# Autodesk Inventor assembly: Right_Upper_Engine_Mount_Rod_Assembly_V1
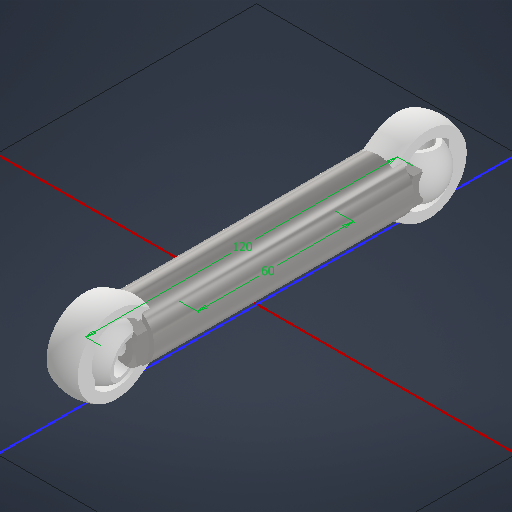
[picture p0: Inventor's stored thumbnail of the model, 512x512]
Saved by Autodesk Inventor 2026.1 (Build 301233000, 233)
## iProperties
Created: 2026-07-28
Part Number: Right_Upper_Engine_Mount_Rod_Assembly_V1
Document SubType Name: Assembly
Designer: share
_SolveAssemblyDoc: Frame Generator Solve Assembly
_Version: 15.0.0
Author: share
## iProperties of the stored document MemberDocs/xWu1g1ya3Psmt1s4v2xjpsksqJb
_SolveAssemblyDoc: Frame Generator Solve Assembly
_Version: 15.0.0
Created: 2026-07-28
Part Number: Right_Upper_Engine_Mount_Rod_Assembly_V1
Document SubType Name: Assembly
Designer: share
Author: share
## Documents named in this file (5)
- C:\Users\share\OneDrive\Documents\Personal Projects\GOGO Kart\CAD\GOGO_KART_FSAE\Drivetrain\Right_Upper_Engine_Mount_Rod_Assembly_V1.iam
- C:\Users\share\OneDrive\Documents\Personal Projects\GOGO Kart\CAD\GOGO_KART_FSAE\Drivetrain\Right_Upper_Engine_Mount_Rod_V1.ipt
- C:\Users\share\OneDrive\Documents\Personal Projects\GOGO Kart\CAD\GOGO_KART_FSAE\Drivetrain\Engine Mount Frame Members\Frame 1785265884395.iam
- C:\Users\share\OneDrive\Documents\Inventor\Content Center Files\R2026\en-US\ISO 8675(2)\ISO 8675 - M12 x 1.5 - ISO.ipt
- C:\Users\share\OneDrive\Documents\Personal Projects\GOGO Kart\CAD\GOGO_KART_FSAE\Suspension\Suspension Arms\Suspension Rod Ends\5-8 Rod End Assembly.iam
## Components (6 placed, 4 different names)
1. Right_Upper_Engine_Mount_Rod_V1:1 — Flush:1, Flush:2, Flush:3, Mate:3, Mate:4
2. Frame 1785265884395:1 [sub-assembly] — Insert:1, Insert:2, Mate:1, Mate:2
3. ISO 8675 M12 x 1.5:1 — Insert:1
4. ISO 8675 M12 x 1.5:2 — Insert:2
5. 5-8 Rod End Assembly:1 [sub-assembly] — Mate:1, Mate:3, Mate:5
6. 5-8 Rod End Assembly:2 [sub-assembly] — Mate:2, Mate:4, Mate:6
## Relationships (11: Mate 6, Flush 3, Insert 2)
- Flush:1: Right_Upper_Engine_Mount_Rod_V1:1
- Flush:2: Right_Upper_Engine_Mount_Rod_V1:1
- Flush:3: Right_Upper_Engine_Mount_Rod_V1:1
- Insert:1: Frame 1785265884395:1 ↔ ISO 8675 M12 x 1.5:1
- Insert:2: Frame 1785265884395:1 ↔ ISO 8675 M12 x 1.5:2
- Mate:1: Frame 1785265884395:1 ↔ 5-8 Rod End Assembly:1
- Mate:2: Frame 1785265884395:1 ↔ 5-8 Rod End Assembly:2
- Mate:3: Right_Upper_Engine_Mount_Rod_V1:1 ↔ 5-8 Rod End Assembly:1
- Mate:4: Right_Upper_Engine_Mount_Rod_V1:1 ↔ 5-8 Rod End Assembly:2
- Mate:5: 5-8 Rod End Assembly:1
- Mate:6: 5-8 Rod End Assembly:2
